# Autodesk Inventor assembly: XCarriage
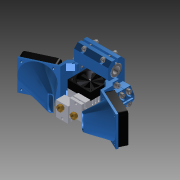
[picture p0: Inventor's stored thumbnail of the model, 180x180]
Saved by Autodesk Inventor 2015 SP1 (Build 190203100, 203)
## iProperties
Created: 2014-12-10
Part Number: XCarriage
Document SubType Name: Assembly
Designer: Jack
Mass: 248.132 g
Surface Area: 960.041 cm^2
Volume: 117.803 cm^3
Density: 2.10633 g/cm^3
Author: Jack
Title: X Carriage
## Documents named in this file (14)
- C:\Users\Jack\ownCloud\Projects\CrossBot\InventorModel\XAxis\XCarriage.iam
- C:\Users\Jack\ownCloud\Projects\CrossBot\InventorModel\HotEnds\E3DChimera\E3DChimera.iam
- C:\Users\Jack\ownCloud\Projects\CrossBot\InventorModel\Electronics\EndStops\EndStopOptical.ipt
- C:\Users\Jack\ownCloud\Projects\CrossBot\InventorModel\XAxis\XCarriageBeltClipRound.ipt
- C:\Users\Jack\ownCloud\Projects\CrossBot\InventorModel\Hardware\Nuts\Nut3.ipt
- C:\Users\Jack\ownCloud\Projects\CrossBot\InventorModel\Hardware\BoltWashers\BoltWasher3\BoltWasher3x16.iam
- C:\Users\Jack\ownCloud\Projects\CrossBot\InventorModel\Hardware\Bearing\BearingLinear\BearingLinearLMUW8.ipt
- C:\Users\Jack\ownCloud\Projects\CrossBot\InventorModel\XAxis\ChimeraXCarriage6.ipt
- C:\Users\Jack\ownCloud\Projects\CrossBot\InventorModel\Hardware\Bolts\SHCS\SHCS3\SHCS3x10.ipt
- C:\Users\Jack\ownCloud\Projects\CrossBot\InventorModel\Electronics\Fans\Fan40mm.ipt
- C:\Users\Jack\ownCloud\Projects\CrossBot\InventorModel\Hardware\BoltWashers\BoltWasher3\BoltWasher3x10.iam
- C:\Users\Jack\ownCloud\Projects\CrossBot\InventorModel\XAxis\ChimeraXCarriage5FanDuct2.ipt
- C:\Users\Jack\ownCloud\Projects\CrossBot\InventorModel\XAxis\ChimeraXCarriage5FanDuct2Mirrored.ipt
- C:\Users\Jack\ownCloud\Projects\CrossBot\InventorModel\Hardware\BoltWashers\BoltWasher3\BoltWasher3x8.iam
## Components (52 placed, 13 different names)
1. E3DChimera:1 [sub-assembly] — Mate:145, Mate:146, Mate:147, Mate:148
2. EndStopOptical:1 — Mate:192, Mate:195, Mate:196, Mate:197, Mate:198
3. XCarriageBeltClipRound:1 — Mate:41, Mate:43, Mate:53, Mate:56, Mate:183
4. XCarriageBeltClipRound:2 — Mate:42, Mate:44, Mate:54, Mate:55, Mate:184
5. XCarriageBeltClipRound:3 — Mate:45, Mate:47, Mate:49, Mate:51, Mate:185
6. XCarriageBeltClipRound:4 — Mate:46, Mate:48, Mate:50, Mate:52, Mate:186
7. BearingLinearLMUW8:1 — Mate:166, Flush:2
8. BearingLinearLMUW8:2 — Mate:165, Flush:1
9. ChimeraXCarriage6:1 — Mate:145, Mate:146, Mate:147, Mate:148, Mate:149, Mate:150, Mate:151, Mate:152, Mate:153, Mate:154, Mate:155, Mate:156, Angle:1, Mate:158, Angle:2, Mate:160, Mate:163, Mate:164, Angle:3, Angle:4, Mate:165, Flush:1, Mate:166, Flush:2, Mate:167, Mate:168, Mate:169, Mate:170, Mate:171, Mate:172, Mate:173, Mate:174, Mate:175, Mate:176, Mate:177, Mate:178, Mate:179, Mate:180, Mate:181, Mate:182, Angle:5, Angle:6, Angle:7, Angle:8, Angle:9, Angle:10, Angle:11, Angle:12, Mate:183, Mate:184, Mate:185, Mate:186, Mate:192, Mate:193, Mate:194, Angle:13, Angle:14, Mate:199, Mate:200, Mate:221, Mate:222, Angle:15, Angle:16, Mate:223, Mate:224, Angle:17, Angle:18, Mate:226, Mate:227, Mate:230, Mate:238, Mate:239, Mate:240, Mate:244, Mate:245, Mate:246, Mate:247, Mate:248, Mate:249
10. ChimeraXCarriage5FanDuct2:1 — Mate:225, Mate:226, Mate:227, Mate:228, Mate:229, Mate:231, Mate:232, Mate:233
11. ChimeraXCarriage5FanDuct2Mirrored:1 — Mate:234, Mate:235, Mate:236, Mate:237, Mate:238, Mate:241, Mate:242, Mate:243
12. BoltWasher3x8:1 [sub-assembly] — Mate:246, Mate:248
13. BoltWasher3x8:2 [sub-assembly] — Mate:245, Mate:249
14. BoltWasher3x8:3 [sub-assembly] — Mate:244, Mate:247
15. Fan40mm:3 — Mate:231, Mate:232, Mate:233
16. Fan40mm:2 — Mate:241, Mate:242, Mate:243
17. BoltWasher3x16:10 [sub-assembly] — Mate:150, Mate:156, Mate:157
18. BoltWasher3x16:9 [sub-assembly] — Mate:149, Mate:155, Mate:159
19. BoltWasher3x16:12 [sub-assembly] — Mate:152, Mate:154, Mate:162
20. BoltWasher3x16:11 [sub-assembly] — Mate:151, Mate:153, Mate:161
21. Nut3:12 — Mate:162, Mate:164, Angle:3
22. Nut3:13 — Mate:161, Mate:163, Angle:4
23. Nut3:9 — Mate:157, Angle:1, Mate:158
24. Nut3:10 — Mate:159, Angle:2, Mate:160
25. BoltWasher3x16:1 [sub-assembly] — Mate:42, Mate:55, Mate:130, Mate:181
26. BoltWasher3x16:2 [sub-assembly] — Mate:41, Mate:56, Mate:128, Mate:180
27. BoltWasher3x16:3 [sub-assembly] — Mate:43, Mate:53, Mate:127, Mate:179
28. BoltWasher3x16:4 [sub-assembly] — Mate:44, Mate:54, Mate:129, Mate:182
29. BoltWasher3x16:5 [sub-assembly] — Mate:45, Mate:49, Mate:142, Mate:176
30. BoltWasher3x16:6 [sub-assembly] — Mate:46, Mate:50, Mate:144, Mate:177
31. BoltWasher3x16:7 [sub-assembly] — Mate:47, Mate:51, Mate:141, Mate:175
32. BoltWasher3x16:8 [sub-assembly] — Mate:48, Mate:52, Mate:143, Mate:178
33. Nut3:1 — Mate:141, Mate:173, Angle:12
34. Nut3:2 — Mate:143, Mate:172, Angle:11
35. Nut3:3 — Mate:127, Mate:167, Angle:6
36. Nut3:4 — Mate:129, Mate:168, Angle:5
37. Nut3:5 — Mate:142, Mate:174, Angle:10
38. Nut3:6 — Mate:144, Mate:171, Angle:9
39. Nut3:7 — Mate:128, Mate:170, Angle:7
40. Nut3:8 — Mate:130, Mate:169, Angle:8
41. Nut3:17 — Mate:218, Mate:224, Angle:17
42. BoltWasher3x10:3 [sub-assembly] — Mate:218, Mate:225, Mate:228, Mate:230
43. BoltWasher3x10:4 [sub-assembly] — Mate:217, Mate:229
44. Nut3:19 — Mate:217, Mate:223, Angle:18
45. Nut3:18 — Mate:219, Mate:222, Angle:15
46. BoltWasher3x10:2 [sub-assembly] — Mate:219, Mate:234, Mate:237, Mate:239
47. BoltWasher3x10:1 [sub-assembly] — Mate:220, Mate:235, Mate:236, Mate:240
48. Nut3:20 — Mate:220, Mate:221, Angle:16
49. SHCS3x10:2 — Mate:196, Mate:197, Mate:200
50. SHCS3x10:1 — Mate:195, Mate:198, Mate:199
51. Nut3:15 — Mate:194, Angle:13
52. Nut3:16 — Mate:193, Angle:14
## Relationships (128: Mate 108, Angle 18, Flush 2)
- Mate:41: XCarriageBeltClipRound:1 ↔ BoltWasher3x16:2
- Mate:42: XCarriageBeltClipRound:2 ↔ BoltWasher3x16:1
- Mate:43: XCarriageBeltClipRound:1 ↔ BoltWasher3x16:3
- Mate:44: XCarriageBeltClipRound:2 ↔ BoltWasher3x16:4
- Mate:45: XCarriageBeltClipRound:3 ↔ BoltWasher3x16:5
- Mate:46: XCarriageBeltClipRound:4 ↔ BoltWasher3x16:6
- Mate:47: XCarriageBeltClipRound:3 ↔ BoltWasher3x16:7
- Mate:48: XCarriageBeltClipRound:4 ↔ BoltWasher3x16:8
- Mate:49: XCarriageBeltClipRound:3 ↔ BoltWasher3x16:5
- Mate:50: XCarriageBeltClipRound:4 ↔ BoltWasher3x16:6
- Mate:51: XCarriageBeltClipRound:3 ↔ BoltWasher3x16:7
- Mate:52: XCarriageBeltClipRound:4 ↔ BoltWasher3x16:8
- Mate:53: XCarriageBeltClipRound:1 ↔ BoltWasher3x16:3
- Mate:54: XCarriageBeltClipRound:2 ↔ BoltWasher3x16:4
- Mate:55: XCarriageBeltClipRound:2 ↔ BoltWasher3x16:1
- Mate:56: XCarriageBeltClipRound:1 ↔ BoltWasher3x16:2
- Mate:127: BoltWasher3x16:3 ↔ Nut3:3
- Mate:128: BoltWasher3x16:2 ↔ Nut3:7
- Mate:129: BoltWasher3x16:4 ↔ Nut3:4
- Mate:130: BoltWasher3x16:1 ↔ Nut3:8
- Mate:141: BoltWasher3x16:7 ↔ Nut3:1
- Mate:142: BoltWasher3x16:5 ↔ Nut3:5
- Mate:143: BoltWasher3x16:8 ↔ Nut3:2
- Mate:144: BoltWasher3x16:6 ↔ Nut3:6
- Mate:145: E3DChimera:1 ↔ ChimeraXCarriage6:1
- Mate:146: E3DChimera:1 ↔ ChimeraXCarriage6:1
- Mate:147: E3DChimera:1 ↔ ChimeraXCarriage6:1
- Mate:148: E3DChimera:1 ↔ ChimeraXCarriage6:1
- Mate:149: ChimeraXCarriage6:1 ↔ BoltWasher3x16:9
- Mate:150: ChimeraXCarriage6:1 ↔ BoltWasher3x16:10
- Mate:151: ChimeraXCarriage6:1 ↔ BoltWasher3x16:11
- Mate:152: ChimeraXCarriage6:1 ↔ BoltWasher3x16:12
- Mate:153: ChimeraXCarriage6:1 ↔ BoltWasher3x16:11
- Mate:154: ChimeraXCarriage6:1 ↔ BoltWasher3x16:12
- Mate:155: ChimeraXCarriage6:1 ↔ BoltWasher3x16:9
- Mate:156: ChimeraXCarriage6:1 ↔ BoltWasher3x16:10
- Mate:157: BoltWasher3x16:10 ↔ Nut3:9
- Angle:1 (0 deg): ChimeraXCarriage6:1 ↔ Nut3:9
- Mate:158: ChimeraXCarriage6:1 ↔ Nut3:9
- Mate:159: BoltWasher3x16:9 ↔ Nut3:10
- Angle:2 (0 deg): ChimeraXCarriage6:1 ↔ Nut3:10
- Mate:160: ChimeraXCarriage6:1 ↔ Nut3:10
- Mate:161: BoltWasher3x16:11 ↔ Nut3:13
- Mate:162: BoltWasher3x16:12 ↔ Nut3:12
- Mate:163: ChimeraXCarriage6:1 ↔ Nut3:13
- Mate:164: ChimeraXCarriage6:1 ↔ Nut3:12
- Angle:3 (0 deg): ChimeraXCarriage6:1 ↔ Nut3:12
- Angle:4 (0 deg): ChimeraXCarriage6:1 ↔ Nut3:13
- Mate:165: BearingLinearLMUW8:2 ↔ ChimeraXCarriage6:1
- Flush:1: BearingLinearLMUW8:2 ↔ ChimeraXCarriage6:1
- Mate:166: BearingLinearLMUW8:1 ↔ ChimeraXCarriage6:1
- Flush:2: BearingLinearLMUW8:1 ↔ ChimeraXCarriage6:1
- Mate:167: ChimeraXCarriage6:1 ↔ Nut3:3
- Mate:168: ChimeraXCarriage6:1 ↔ Nut3:4
- Mate:169: ChimeraXCarriage6:1 ↔ Nut3:8
- Mate:170: ChimeraXCarriage6:1 ↔ Nut3:7
- Mate:171: ChimeraXCarriage6:1 ↔ Nut3:6
- Mate:172: ChimeraXCarriage6:1 ↔ Nut3:2
- Mate:173: ChimeraXCarriage6:1 ↔ Nut3:1
- Mate:174: ChimeraXCarriage6:1 ↔ Nut3:5
- Mate:175: ChimeraXCarriage6:1 ↔ BoltWasher3x16:7
- Mate:176: ChimeraXCarriage6:1 ↔ BoltWasher3x16:5
- Mate:177: ChimeraXCarriage6:1 ↔ BoltWasher3x16:6
- Mate:178: ChimeraXCarriage6:1 ↔ BoltWasher3x16:8
- Mate:179: ChimeraXCarriage6:1 ↔ BoltWasher3x16:3
- Mate:180: ChimeraXCarriage6:1 ↔ BoltWasher3x16:2
- Mate:181: ChimeraXCarriage6:1 ↔ BoltWasher3x16:1
- Mate:182: ChimeraXCarriage6:1 ↔ BoltWasher3x16:4
- Angle:5 (0 deg): ChimeraXCarriage6:1 ↔ Nut3:4
- Angle:6 (0 deg): ChimeraXCarriage6:1 ↔ Nut3:3
- Angle:7 (0 deg): ChimeraXCarriage6:1 ↔ Nut3:7
- Angle:8 (0 deg): ChimeraXCarriage6:1 ↔ Nut3:8
- Angle:9 (0 deg): ChimeraXCarriage6:1 ↔ Nut3:6
- Angle:10 (0 deg): ChimeraXCarriage6:1 ↔ Nut3:5
- Angle:11 (0 deg): ChimeraXCarriage6:1 ↔ Nut3:2
- Angle:12 (0 deg): ChimeraXCarriage6:1 ↔ Nut3:1
- Mate:183: XCarriageBeltClipRound:1 ↔ ChimeraXCarriage6:1
- Mate:184: XCarriageBeltClipRound:2 ↔ ChimeraXCarriage6:1
- Mate:185: XCarriageBeltClipRound:3 ↔ ChimeraXCarriage6:1
- Mate:186: XCarriageBeltClipRound:4 ↔ ChimeraXCarriage6:1
- Mate:192: EndStopOptical:1 ↔ ChimeraXCarriage6:1
- Mate:193: ChimeraXCarriage6:1 ↔ Nut3:16
- Mate:194: ChimeraXCarriage6:1 ↔ Nut3:15
- Angle:13 (0 deg): ChimeraXCarriage6:1 ↔ Nut3:15
- Angle:14 (0 deg): ChimeraXCarriage6:1 ↔ Nut3:16
- Mate:195: EndStopOptical:1 ↔ SHCS3x10:1
- Mate:196: EndStopOptical:1 ↔ SHCS3x10:2
- Mate:197: EndStopOptical:1 ↔ SHCS3x10:2
- Mate:198: EndStopOptical:1 ↔ SHCS3x10:1
- Mate:199: ChimeraXCarriage6:1 ↔ SHCS3x10:1
- Mate:200: ChimeraXCarriage6:1 ↔ SHCS3x10:2
- Mate:217: BoltWasher3x10:4 ↔ Nut3:19
- Mate:218: Nut3:17 ↔ BoltWasher3x10:3
- Mate:219: Nut3:18 ↔ BoltWasher3x10:2
- Mate:220: BoltWasher3x10:1 ↔ Nut3:20
- Mate:221: ChimeraXCarriage6:1 ↔ Nut3:20
- Mate:222: ChimeraXCarriage6:1 ↔ Nut3:18
- Angle:15 (0 deg): ChimeraXCarriage6:1 ↔ Nut3:18
- Angle:16 (0 deg): ChimeraXCarriage6:1 ↔ Nut3:20
- Mate:223: ChimeraXCarriage6:1 ↔ Nut3:19
- Mate:224: ChimeraXCarriage6:1 ↔ Nut3:17
- Angle:17 (0 deg): ChimeraXCarriage6:1 ↔ Nut3:17
- Angle:18 (0 deg): ChimeraXCarriage6:1 ↔ Nut3:19
- Mate:225: ChimeraXCarriage5FanDuct2:1 ↔ BoltWasher3x10:3
- Mate:226: ChimeraXCarriage6:1 ↔ ChimeraXCarriage5FanDuct2:1
- Mate:227: ChimeraXCarriage6:1 ↔ ChimeraXCarriage5FanDuct2:1
- Mate:228: ChimeraXCarriage5FanDuct2:1 ↔ BoltWasher3x10:3
- Mate:229: ChimeraXCarriage5FanDuct2:1 ↔ BoltWasher3x10:4
- Mate:230: ChimeraXCarriage6:1 ↔ BoltWasher3x10:3
- Mate:231: ChimeraXCarriage5FanDuct2:1 ↔ Fan40mm:3
- Mate:232: ChimeraXCarriage5FanDuct2:1 ↔ Fan40mm:3
- Mate:233: ChimeraXCarriage5FanDuct2:1 ↔ Fan40mm:3
- Mate:234: ChimeraXCarriage5FanDuct2Mirrored:1 ↔ BoltWasher3x10:2
- Mate:235: ChimeraXCarriage5FanDuct2Mirrored:1 ↔ BoltWasher3x10:1
- Mate:236: ChimeraXCarriage5FanDuct2Mirrored:1 ↔ BoltWasher3x10:1
- Mate:237: ChimeraXCarriage5FanDuct2Mirrored:1 ↔ BoltWasher3x10:2
- Mate:238: ChimeraXCarriage6:1 ↔ ChimeraXCarriage5FanDuct2Mirrored:1
- Mate:239: ChimeraXCarriage6:1 ↔ BoltWasher3x10:2
- Mate:240: ChimeraXCarriage6:1 ↔ BoltWasher3x10:1
- Mate:241: ChimeraXCarriage5FanDuct2Mirrored:1 ↔ Fan40mm:2
- Mate:242: ChimeraXCarriage5FanDuct2Mirrored:1 ↔ Fan40mm:2
- Mate:243: ChimeraXCarriage5FanDuct2Mirrored:1 ↔ Fan40mm:2
- Mate:244: ChimeraXCarriage6:1 ↔ BoltWasher3x8:3
- Mate:245: ChimeraXCarriage6:1 ↔ BoltWasher3x8:2
- Mate:246: ChimeraXCarriage6:1 ↔ BoltWasher3x8:1
- Mate:247: ChimeraXCarriage6:1 ↔ BoltWasher3x8:3
- Mate:248: ChimeraXCarriage6:1 ↔ BoltWasher3x8:1
- Mate:249: ChimeraXCarriage6:1 ↔ BoltWasher3x8:2
